# Autodesk Inventor assembly: SKF_UCFL 205
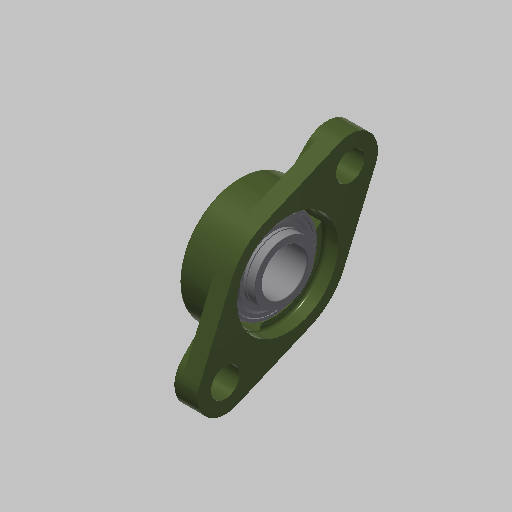
[picture p0: Inventor's stored thumbnail of the model, 512x512]
Saved by Autodesk Inventor 2025.2 (Build 292293000, 293)
## iProperties
Category: PARTsolutions
Company: SKF
Created: 2024-04-15
Part Number: SKF_UCFL 205
Catalog Web Link: www.cadenas.de
Description: AYF_002HC_HH_HY_AYD_001HP-Y-bearing oval flanged units
Vendor: SKF
Document SubType Name: Assembly
Designer: psAdmin
Manufacturer: SKF
Mass: 610 g
Surface Area: 453.005 cm^2
Volume: 85.044 cm^3
Density: 7.17276 g/cm^3
PSOL_IDENT_0: {$CADENAS_DATA/23d-libs/skf/bearings_units_and_housings/bearing_units/ball_bearing_units/y-units/ayf
PSOL_IDENT_1: _002hc_hh_hy_ayd_001hp.prj},205 {VTYP=3D},{STYP=ASSTAB},{NB=SKF_UCFL 205},{LINA=SKF_UCFL 205},{NN=AY
PSOL_IDENT_2: F_002HC_HH_HY_AYD_001HP},{DATE=23.02.2024 07:59:20},{GEOMDATE=22.02.2024 06:03:03},{VERSION=},{LINEI
PSOL_IDENT_3: D=74190},{WBVAR=COVER},{WBNUMERIC=}  {NB=SKF_UCFL 205},{LINA=SKF_UCFL 205},{KT=DUMMY},{DESIGNATION=U
PSOL_IDENT_4: CFL 205},{DAAX=0.000},{COVER=},{D=52.000},{DD=25.0000},{B=34.000},{C=15.000},{PITCH=39.000},{DW=7.93
PSOL_IDENT_5: 8},{DD1=33.700},{DD2=0.000},{A=27.000},{T=35.700},{DAMIN=},{DAA=},{DB1=68},{DB2=},{DB=},{B1=},{J=99}
PSOL_IDENT_6: ,{H=130.000},{L=68.000},{N=16},{SS1=19.700},{DN=6.6},{J6=},{J7=},{R12=1.5},{B3=},{D1=},{K=},{CC1=},{
PSOL_IDENT_7: RG=1/4-28 UNF},{GN=1/4-28 UNF},{LOAD1=14.000},{LOAD2=7.800},{LOAD3=0.335},{SPEED=MIN},{SPEED1=5850},
PSOL_IDENT_8: {II=1},{Z=9},{G2=M6x1},{G=14},{GIN=0.5625000037125},{MASS=0.61},{HOUSING=},{HNEW=FL 205/Y},{HALG=FL
PSOL_IDENT_9: 205/Y},{BNEW=},{BEARING=UC 205},{EC=},{ECX=ECY 205},{ECXX=},{ECXXX=},{ECY=ECY 205},{BS=},{SLEEVE=},{
PSOL_IDENT_10: A1=13},{A2=},{A3=},{A5=20.5},{B4=5.5},{DESIGN=uclf},{SUPPRESSED=unsuppressed},{BRGTYP=BBY_006},{COVE
PSOL_IDENT_11: RALG=  '', 'No End Cover', 'ECY 205', 'ECY 205' },{PPATH=y-bearing_oval_flanged_units_parts/ayf_002h
PSOL_IDENT_12: c_hh_hy_ayd_001hp_asmtpl.prj},{TC=UCFL 205},{SUPHELP=0}
NB: SKF_UCFL 205
NN: AYF_002HC_HH_HY_AYD_001HP
NT: Y-bearing oval flanged units
NBSYN: SKF_$TC.
LINA: SKF_UCFL 205
CATALOG: SKF
DESIGNATION: UCFL 205
COVER: No End Cover
T: 35.7
J: 99
L: 68
LOAD1: 14
LOAD2: 7.8
SPEED1: 5850
BEARING: UC 205
SUPPLIER: SKF
ARTICLENO: SKF_UCFL 205
BOMINFO: SKF_UCFL 205
CREATOR: CADENAS GmbH
Title: SKF_UCFL 205
Author: Cadenas PARTsolutions
Comments: Y-bearing oval flanged units
## Documents named in this file (5)
- C:\Users\phmca\OneDrive\Documentos\TCC\TCC\AIS2023\SKF_UCFL 205.iam
- C:\Users\phmca\OneDrive\Documentos\TCC\TCC\AIS2023\FL 205_Y++35_7_h.ipt
- C:\Users\phmca\OneDrive\Documentos\TCC\TCC\AIS2023\1_4-28 UNF.ipt
- C:\Users\phmca\OneDrive\Documentos\TCC\TCC\AIS2023\UC 205+33_7_b.ipt
- C:\Users\phmca\OneDrive\Documentos\TCC\TCC\AIS2023\ucfl-IEC_BBY_006-25-34--52-15-39-7_938.ipt
## Components (12 placed, 4 different names)
1. FL 205_Y++35_7_h:1 — gn_XY@1 <-> gn_XY@2, gn_Z@1 <-> gn_Z@2, gn_YZ@1 <-> gn_YZ@2, Coincidente:21, Coincidente:22
2. 1_4-28 UNF:1 — gn_XY@1 <-> gn_XY@2, gn_Z@1 <-> gn_Z@2, gn_YZ@1 <-> gn_YZ@2
3. UC 205+33_7_b:1 — ball_1_XY@3 <-> ball_XY@4, ball_1_Z@3 <-> ball_Z@4, ball_1_YZ@3 <-> ball_YZ@4, ball_2_XY@3 <-> ball_XY@5, ball_2_Z@3 <-> ball_Z@5, ball_2_YZ@3 <-> ball_YZ@5, ball_3_XY@3 <-> ball_XY@6, ball_3_Z@3 <-> ball_Z@6, ball_3_YZ@3 <-> ball_YZ@6, ball_4_XY@3 <-> ball_XY@7, ball_4_Z@3 <-> ball_Z@7, ball_4_YZ@3 <-> ball_YZ@7, ball_5_XY@3 <-> ball_XY@8, ball_5_Z@3 <-> ball_Z@8, ball_5_YZ@3 <-> ball_YZ@8, ball_6_XY@3 <-> ball_XY@9, ball_6_Z@3 <-> ball_Z@9, ball_6_YZ@3 <-> ball_YZ@9, ball_7_XY@3 <-> ball_XY@10, ball_7_Z@3 <-> ball_Z@10, ball_7_YZ@3 <-> ball_YZ@10, ball_8_XY@3 <-> ball_XY@11, ball_8_Z@3 <-> ball_Z@11, ball_8_YZ@3 <-> ball_YZ@11, ball_9_XY@3 <-> ball_XY@12, ball_9_Z@3 <-> ball_Z@12, ball_9_YZ@3 <-> ball_YZ@12
4. ucfl-IEC_BBY_006-25-34--52-15-39-7_938:1 — ball_1_XY@3 <-> ball_XY@4, ball_1_Z@3 <-> ball_Z@4, ball_1_YZ@3 <-> ball_YZ@4
5. ucfl-IEC_BBY_006-25-34--52-15-39-7_938:2 — ball_2_XY@3 <-> ball_XY@5, ball_2_Z@3 <-> ball_Z@5, ball_2_YZ@3 <-> ball_YZ@5
6. ucfl-IEC_BBY_006-25-34--52-15-39-7_938:3 — ball_3_XY@3 <-> ball_XY@6, ball_3_Z@3 <-> ball_Z@6, ball_3_YZ@3 <-> ball_YZ@6
7. ucfl-IEC_BBY_006-25-34--52-15-39-7_938:4 — ball_4_XY@3 <-> ball_XY@7, ball_4_Z@3 <-> ball_Z@7, ball_4_YZ@3 <-> ball_YZ@7
8. ucfl-IEC_BBY_006-25-34--52-15-39-7_938:5 — ball_5_XY@3 <-> ball_XY@8, ball_5_Z@3 <-> ball_Z@8, ball_5_YZ@3 <-> ball_YZ@8
9. ucfl-IEC_BBY_006-25-34--52-15-39-7_938:6 — ball_6_XY@3 <-> ball_XY@9, ball_6_Z@3 <-> ball_Z@9, ball_6_YZ@3 <-> ball_YZ@9
10. ucfl-IEC_BBY_006-25-34--52-15-39-7_938:7 — ball_7_XY@3 <-> ball_XY@10, ball_7_Z@3 <-> ball_Z@10, ball_7_YZ@3 <-> ball_YZ@10
11. ucfl-IEC_BBY_006-25-34--52-15-39-7_938:8 — ball_8_XY@3 <-> ball_XY@11, ball_8_Z@3 <-> ball_Z@11, ball_8_YZ@3 <-> ball_YZ@11
12. ucfl-IEC_BBY_006-25-34--52-15-39-7_938:9 — ball_9_XY@3 <-> ball_XY@12, ball_9_Z@3 <-> ball_Z@12, ball_9_YZ@3 <-> ball_YZ@12
## Relationships (34: Mate 24, Angle 10)
- gn_XY@1 <-> gn_XY@2 [Mate]: FL 205_Y++35_7_h:1 ↔ 1_4-28 UNF:1
- gn_Z@1 <-> gn_Z@2 [Mate]: FL 205_Y++35_7_h:1 ↔ 1_4-28 UNF:1
- gn_YZ@1 <-> gn_YZ@2 [Angle] (110 deg): FL 205_Y++35_7_h:1 ↔ 1_4-28 UNF:1
- ball_1_XY@3 <-> ball_XY@4 [Mate]: UC 205+33_7_b:1 ↔ ucfl-IEC_BBY_006-25-34--52-15-39-7_938:1
- ball_1_Z@3 <-> ball_Z@4 [Mate]: UC 205+33_7_b:1 ↔ ucfl-IEC_BBY_006-25-34--52-15-39-7_938:1
- ball_1_YZ@3 <-> ball_YZ@4 [Angle] (0 deg): UC 205+33_7_b:1 ↔ ucfl-IEC_BBY_006-25-34--52-15-39-7_938:1
- ball_2_XY@3 <-> ball_XY@5 [Mate]: UC 205+33_7_b:1 ↔ ucfl-IEC_BBY_006-25-34--52-15-39-7_938:2
- ball_2_Z@3 <-> ball_Z@5 [Mate]: UC 205+33_7_b:1 ↔ ucfl-IEC_BBY_006-25-34--52-15-39-7_938:2
- ball_2_YZ@3 <-> ball_YZ@5 [Angle] (0 deg): UC 205+33_7_b:1 ↔ ucfl-IEC_BBY_006-25-34--52-15-39-7_938:2
- ball_3_XY@3 <-> ball_XY@6 [Mate]: UC 205+33_7_b:1 ↔ ucfl-IEC_BBY_006-25-34--52-15-39-7_938:3
- ball_3_Z@3 <-> ball_Z@6 [Mate]: UC 205+33_7_b:1 ↔ ucfl-IEC_BBY_006-25-34--52-15-39-7_938:3
- ball_3_YZ@3 <-> ball_YZ@6 [Angle] (0 deg): UC 205+33_7_b:1 ↔ ucfl-IEC_BBY_006-25-34--52-15-39-7_938:3
- ball_4_XY@3 <-> ball_XY@7 [Mate]: UC 205+33_7_b:1 ↔ ucfl-IEC_BBY_006-25-34--52-15-39-7_938:4
- ball_4_Z@3 <-> ball_Z@7 [Mate]: UC 205+33_7_b:1 ↔ ucfl-IEC_BBY_006-25-34--52-15-39-7_938:4
- ball_4_YZ@3 <-> ball_YZ@7 [Angle] (0 deg): UC 205+33_7_b:1 ↔ ucfl-IEC_BBY_006-25-34--52-15-39-7_938:4
- ball_5_XY@3 <-> ball_XY@8 [Mate]: UC 205+33_7_b:1 ↔ ucfl-IEC_BBY_006-25-34--52-15-39-7_938:5
- ball_5_Z@3 <-> ball_Z@8 [Mate]: UC 205+33_7_b:1 ↔ ucfl-IEC_BBY_006-25-34--52-15-39-7_938:5
- ball_5_YZ@3 <-> ball_YZ@8 [Angle] (0 deg): UC 205+33_7_b:1 ↔ ucfl-IEC_BBY_006-25-34--52-15-39-7_938:5
- ball_6_XY@3 <-> ball_XY@9 [Mate]: UC 205+33_7_b:1 ↔ ucfl-IEC_BBY_006-25-34--52-15-39-7_938:6
- ball_6_Z@3 <-> ball_Z@9 [Mate]: UC 205+33_7_b:1 ↔ ucfl-IEC_BBY_006-25-34--52-15-39-7_938:6
- ball_6_YZ@3 <-> ball_YZ@9 [Angle] (0 deg): UC 205+33_7_b:1 ↔ ucfl-IEC_BBY_006-25-34--52-15-39-7_938:6
- ball_7_XY@3 <-> ball_XY@10 [Mate]: UC 205+33_7_b:1 ↔ ucfl-IEC_BBY_006-25-34--52-15-39-7_938:7
- ball_7_Z@3 <-> ball_Z@10 [Mate]: UC 205+33_7_b:1 ↔ ucfl-IEC_BBY_006-25-34--52-15-39-7_938:7
- ball_7_YZ@3 <-> ball_YZ@10 [Angle] (0 deg): UC 205+33_7_b:1 ↔ ucfl-IEC_BBY_006-25-34--52-15-39-7_938:7
- ball_8_XY@3 <-> ball_XY@11 [Mate]: UC 205+33_7_b:1 ↔ ucfl-IEC_BBY_006-25-34--52-15-39-7_938:8
- ball_8_Z@3 <-> ball_Z@11 [Mate]: UC 205+33_7_b:1 ↔ ucfl-IEC_BBY_006-25-34--52-15-39-7_938:8
- ball_8_YZ@3 <-> ball_YZ@11 [Angle] (0 deg): UC 205+33_7_b:1 ↔ ucfl-IEC_BBY_006-25-34--52-15-39-7_938:8
- ball_9_XY@3 <-> ball_XY@12 [Mate]: UC 205+33_7_b:1 ↔ ucfl-IEC_BBY_006-25-34--52-15-39-7_938:9
- ball_9_Z@3 <-> ball_Z@12 [Mate]: UC 205+33_7_b:1 ↔ ucfl-IEC_BBY_006-25-34--52-15-39-7_938:9
- ball_9_YZ@3 <-> ball_YZ@12 [Angle] (0 deg): UC 205+33_7_b:1 ↔ ucfl-IEC_BBY_006-25-34--52-15-39-7_938:9
- Coincidente:21 [Mate]: FL 205_Y++35_7_h:1
- Coincidente:22 [Mate]: FL 205_Y++35_7_h:1
- Coincidente:23 [Mate]
- Coincidente:24 [Mate]
